# Autodesk Inventor assembly: LinearBearing8mm
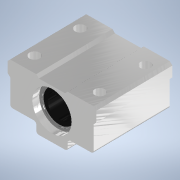
[picture p0: Inventor's stored thumbnail of the model, 180x180]
Saved by Autodesk Inventor 2020.2 (Build 242310000, 310)
## iProperties
Created: 2020-07-30
Part Number: LinearBearing8mm
Document SubType Name: Assembly
Designer: JK
Author: JK
## Documents named in this file (3)
- C:\Users\JK\Documents\Inventor\Anet Upgrade\LinearBearing8mm.iam
- C:\Users\JK\Documents\Inventor\Anet Upgrade\LM8UU.ipt
- C:\Users\JK\Documents\Inventor\Anet Upgrade\LM8UU 8mm Linear Bearing.ipt
## Components (2 placed, 2 different names)
1. LM8UU:1
2. LM8UU 8mm Linear Bearing:1
## Relationships (2: Mate 1, Flush 1)
- [Mate]: LM8UU:1 ↔ LM8UU 8mm Linear Bearing:1
- [Flush] (2.5 mm): LM8UU:1 ↔ LM8UU 8mm Linear Bearing:1
